# Autodesk Inventor assembly: Ensamble NotAFarmBot2
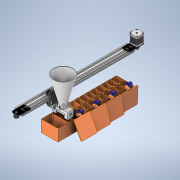
[picture p0: Inventor's stored thumbnail of the model, 180x180]
Saved by Autodesk Inventor 2022 (Build 260153000, 153)
## iProperties
Created: 2020-07-22
Part Number: Ensamble NotAFarmBot2
Document SubType Name: Assembly
Designer: juanp
Mass: 2768.3 g
Surface Area: 9738.48 cm^2
Volume: 1823.12 cm^3
Density: 1.51844 g/cm^3
Author: juanp
## Documents named in this file (24)
- C:\Users\juanp\OneDrive - Universidad de los andes\Uniandes\Robocol\EVA\V0  (Antiguo)\Ensamble NotAFarmBot2.iam
- C:\Users\juanp\OneDrive - Universidad de los andes\Uniandes\Robocol\EVA\V0  (Antiguo)\VSLOT 2040 Extrusion.ipt
- C:\Users\juanp\OneDrive - Universidad de los andes\Uniandes\Robocol\EVA\V0  (Antiguo)\Double Tee Nut.ipt
- C:\Users\juanp\OneDrive - Universidad de los andes\Uniandes\Robocol\EVA\V0  (Antiguo)\GT2_30T_5_6.ipt
- C:\Users\juanp\OneDrive - Universidad de los andes\Uniandes\Robocol\EVA\V0  (Antiguo)\Idler Pulley Plate.ipt
- C:\Users\juanp\OneDrive - Universidad de los andes\Uniandes\Robocol\EVA\V0  (Antiguo)\Motor Mount Plate Nema 17.ipt
- C:\Users\juanp\OneDrive - Universidad de los andes\Uniandes\Robocol\EVA\V0  (Antiguo)\NEMA 17 simple\M1173041- NEMA 17.ipt
- C:\Users\juanp\OneDrive - Universidad de los andes\Uniandes\Robocol\EVA\V0  (Antiguo)\Gantry\Inventor\20mm Gantry Set.iam
- C:\Users\juanp\OneDrive - Universidad de los andes\Uniandes\Robocol\EVA\V0  (Antiguo)\3mm Spacer.ipt
- C:\Users\juanp\OneDrive - Universidad de los andes\Uniandes\Robocol\EVA\V0  (Antiguo)\VSLOT Attachments\M5x25 low profile screw.ipt
- C:\Users\juanp\OneDrive - Universidad de los andes\Uniandes\Robocol\EVA\V0  (Antiguo)\VSLOT Attachments\Ball Bearing 625 2RS 5x16x5.ipt
- C:\Users\juanp\OneDrive - Universidad de los andes\Uniandes\Robocol\EVA\V0  (Antiguo)\VSLOT Attachments\1mm 5mm shim.ipt
- C:\Users\juanp\OneDrive - Universidad de los andes\Uniandes\Robocol\EVA\V0  (Antiguo)\VSLOT Attachments\Nylon Spacer 1_8th.ipt
- C:\Users\juanp\OneDrive - Universidad de los andes\Uniandes\Robocol\EVA\V0  (Antiguo)\VSLOT Attachments\idler pulley.ipt
- C:\Users\juanp\OneDrive - Universidad de los andes\Uniandes\Robocol\EVA\V0  (Antiguo)\Gantry\Inventor\M5 Nylock.ipt
- C:\Users\juanp\OneDrive - Universidad de los andes\Uniandes\Robocol\EVA\V0  (Antiguo)\VSLOT Attachments\M5x8 low profile screw.ipt
- C:\Users\juanp\Documents\Inventor\Content Center Files\R2020\en-US\ANSI B18.3.4M(1)\ANSI B18.3.4M - M3 x 0.5 x 8(2).ipt
- C:\Users\juanp\OneDrive - Universidad de los andes\Uniandes\Robocol\EVA\V0  (Antiguo)\Dispensador V2\Ensamble Dispensador V2.iam
- C:\Users\juanp\OneDrive - Universidad de los andes\Uniandes\Robocol\EVA\V0  (Antiguo)\Gantry\Inventor\M5x35 low profile screw.ipt
- C:\Users\juanp\Documents\Inventor\Content Center Files\R2020\en-US\ANSI B18.3.1M(6)\ANSI B18.3.1M - M2x0.4 x 16(1).ipt
- C:\Users\juanp\Documents\Inventor\Content Center Files\R2020\en-US\ANSI B 18.2.4.1 M(1)\ANSI B 18.2.4.1 M - M2 x 0.4Style 1.ipt
- C:\Users\juanp\OneDrive - Universidad de los andes\Uniandes\Robocol\EVA\V0  (Antiguo)\Tapas.ipt
- C:\Users\juanp\OneDrive - Universidad de los andes\Uniandes\Robocol\EVA\V0  (Antiguo)\SERVO\SG90 - Micro Servo 9g - Tower Pro.iam
- C:\Users\juanp\OneDrive - Universidad de los andes\Uniandes\Robocol\EVA\V0  (Antiguo)\Contenedor3.ipt
## Components (44 placed, 23 different names)
1. VSLOT 2040 Extrusion:1 — Angle:5, Angle:6, Tangent:1, Tangent:2, Mate:85, Mate:86, Mate:87, Mate:88, Angle:16, Mate:98, Mate:99, Angle:18, Mate:100, Mate:101, Angle:23, Angle:24, Flush:3, Mate:180
2. Double Tee Nut:1 — Mate:98, Mate:99, Angle:18, Mate:100, Mate:106
3. Double Tee Nut:2 — Mate:85, Mate:86, Mate:87, Mate:93, Angle:16, Mate:94
4. GT2_30T_5_6:2 — Mate:35, Mate:107
5. Idler Pulley Plate:1 — Mate:88, Mate:89, Mate:90, Mate:91, Mate:92, Mate:95, Mate:96, Mate:97, Angle:17
6. Motor Mount Plate Nema 17:1 — Mate:12, Mate:13, Angle:4, Mate:42, Mate:43, Mate:52, Mate:53, Mate:54, Mate:55, Mate:56, Mate:101, Mate:102, Mate:103, Mate:104, Mate:105
7. M1173041- NEMA 17:1 — Mate:12, Mate:13, Angle:4, Mate:48, Mate:49, Mate:50, Mate:51, Mate:107
8. 20mm Gantry Set:1 [sub-assembly] — Angle:5, Angle:6, Tangent:1, Tangent:2, Mate:56, Mate:121, Mate:124, Mate:126
9. M5x25 low profile screw:1 — Mate:27, Mate:28, Mate:29, Mate:31, Mate:46, Mate:96
10. Ball Bearing 625 2RS 5x16x5:1 — Mate:22, Mate:23, Mate:24, Mate:26, Mate:32
11. Ball Bearing 625 2RS 5x16x5:2 — Mate:21, Mate:25, Mate:28
12. 1mm 5mm shim:1 — Mate:29, Mate:47, Mate:97
13. Nylon Spacer 1_8th:1 — Mate:23, Mate:24, Mate:25
14. idler pulley:1 — Mate:21, Mate:22, Mate:26, Mate:27, Mate:35
15. 3mm Spacer:1 — Mate:31, Mate:32, Mate:95
16. M5x8 low profile screw:1 — Mate:42, Mate:102, Mate:104
17. M5x8 low profile screw:2 — Mate:43, Mate:103, Mate:105, Mate:106
18. M5x8 low profile screw:3 — Mate:90, Mate:92, Mate:94
19. M5x8 low profile screw:4 — Mate:89, Mate:91, Mate:93
20. M5 Nylock:1 — Mate:46, Mate:47, Angle:17
21. Broached Hexagon Socket Button Head Cap Screw - Metric M3 x 0.5 x 8:1 — Mate:50, Mate:54
22. Broached Hexagon Socket Button Head Cap Screw - Metric M3 x 0.5 x 8:2 — Mate:51, Mate:55
23. Broached Hexagon Socket Button Head Cap Screw - Metric M3 x 0.5 x 8:3 — Mate:49, Mate:52
24. Broached Hexagon Socket Button Head Cap Screw - Metric M3 x 0.5 x 8:4 — Mate:48, Mate:53
25. Ensamble Dispensador V2:1 [sub-assembly] — Mate:121, Mate:123, Mate:125, Mate:127, Mate:128, Mate:129, Mate:130, Mate:131, Mate:132, Mate:137, Mate:138, Angle:19, Angle:20, Mate:139, Mate:140, Mate:141, Mate:142, Mate:143, Mate:144, Angle:21, Angle:22, Mate:181
26. M5x35 low profile screw:1 — Mate:125, Mate:126, Mate:128
27. M5x35 low profile screw:2 — Mate:123, Mate:124, Mate:127
28. Forged Socket Head Cap Screw - Metric M2x0.4 x 16:1 — Mate:129, Mate:132, Mate:133
29. Forged Socket Head Cap Screw - Metric M2x0.4 x 16:2 — Mate:130, Mate:131, Mate:134
30. Hex Nut Metric M2 x 0.4:1 — Mate:135, Mate:144, Angle:22
31. Hex Nut Metric M2 x 0.4:2 — Mate:136, Mate:143, Angle:21
32. Hex Nut Metric M2 x 0.4:3 — Mate:134, Mate:138, Angle:19
33. Hex Nut Metric M2 x 0.4:4 — Mate:133, Mate:137, Angle:20
34. Forged Socket Head Cap Screw - Metric M2x0.4 x 16:3 — Mate:135, Mate:140, Mate:142
35. Forged Socket Head Cap Screw - Metric M2x0.4 x 16:4 — Mate:136, Mate:139, Mate:141
36. Tapas:1 — Mate:152, Mate:153, Mate:179, Flush:4
37. Tapas:2 — Mate:160, Mate:161, Mate:177, Mate:179
38. SG90 - Micro Servo 9g - Tower Pro:1 [sub-assembly] — Mate:152, Mate:153, Mate:164, Mate:165
39. SG90 - Micro Servo 9g - Tower Pro:2 [sub-assembly] — Mate:160, Mate:161, Mate:166, Mate:167
40. Contenedor3:1 — Angle:23, Angle:24, Mate:164, Mate:165, Mate:166, Mate:167, Mate:172, Mate:173, Mate:174, Mate:175, Flush:3, Flush:4, Mate:180, Mate:181
41. Tapas:3 — Mate:178
42. SG90 - Micro Servo 9g - Tower Pro:3 [sub-assembly] — Mate:172, Mate:173
43. Tapas:4 — Mate:177, Mate:178
44. SG90 - Micro Servo 9g - Tower Pro:4 [sub-assembly] — Mate:174, Mate:175
## Relationships (110: Mate 94, Angle 12, Tangent 2, Flush 2)
- Mate:12: Motor Mount Plate Nema 17:1 ↔ M1173041- NEMA 17:1
- Mate:13: Motor Mount Plate Nema 17:1 ↔ M1173041- NEMA 17:1
- Angle:4 (0 deg): Motor Mount Plate Nema 17:1 ↔ M1173041- NEMA 17:1
- Angle:5 (0 deg): VSLOT 2040 Extrusion:1 ↔ 20mm Gantry Set:1
- Angle:6 (0 deg): VSLOT 2040 Extrusion:1 ↔ 20mm Gantry Set:1
- Tangent:1: VSLOT 2040 Extrusion:1 ↔ 20mm Gantry Set:1
- Tangent:2: VSLOT 2040 Extrusion:1 ↔ 20mm Gantry Set:1
- Mate:21: Ball Bearing 625 2RS 5x16x5:2 ↔ idler pulley:1
- Mate:22: Ball Bearing 625 2RS 5x16x5:1 ↔ idler pulley:1
- Mate:23: Ball Bearing 625 2RS 5x16x5:1 ↔ Nylon Spacer 1_8th:1
- Mate:24: Ball Bearing 625 2RS 5x16x5:1 ↔ Nylon Spacer 1_8th:1
- Mate:25: Ball Bearing 625 2RS 5x16x5:2 ↔ Nylon Spacer 1_8th:1
- Mate:26: Ball Bearing 625 2RS 5x16x5:1 ↔ idler pulley:1
- Mate:27: M5x25 low profile screw:1 ↔ idler pulley:1
- Mate:28: M5x25 low profile screw:1 ↔ Ball Bearing 625 2RS 5x16x5:2
- Mate:29: M5x25 low profile screw:1 ↔ 1mm 5mm shim:1
- Mate:31: M5x25 low profile screw:1 ↔ 3mm Spacer:1
- Mate:32: Ball Bearing 625 2RS 5x16x5:1 ↔ 3mm Spacer:1
- Mate:35: GT2_30T_5_6:2 ↔ idler pulley:1
- Mate:42: Motor Mount Plate Nema 17:1 ↔ M5x8 low profile screw:1
- Mate:43: Motor Mount Plate Nema 17:1 ↔ M5x8 low profile screw:2
- Mate:46: M5x25 low profile screw:1 ↔ M5 Nylock:1
- Mate:47: 1mm 5mm shim:1 ↔ M5 Nylock:1
- Mate:48: M1173041- NEMA 17:1 ↔ Broached Hexagon Socket Button Head Cap Screw - Metric M3 x 0.5 x 8:4
- Mate:49: M1173041- NEMA 17:1 ↔ Broached Hexagon Socket Button Head Cap Screw - Metric M3 x 0.5 x 8:3
- Mate:50: M1173041- NEMA 17:1 ↔ Broached Hexagon Socket Button Head Cap Screw - Metric M3 x 0.5 x 8:1
- Mate:51: M1173041- NEMA 17:1 ↔ Broached Hexagon Socket Button Head Cap Screw - Metric M3 x 0.5 x 8:2
- Mate:52: Motor Mount Plate Nema 17:1 ↔ Broached Hexagon Socket Button Head Cap Screw - Metric M3 x 0.5 x 8:3
- Mate:53: Motor Mount Plate Nema 17:1 ↔ Broached Hexagon Socket Button Head Cap Screw - Metric M3 x 0.5 x 8:4
- Mate:54: Motor Mount Plate Nema 17:1 ↔ Broached Hexagon Socket Button Head Cap Screw - Metric M3 x 0.5 x 8:1
- Mate:55: Motor Mount Plate Nema 17:1 ↔ Broached Hexagon Socket Button Head Cap Screw - Metric M3 x 0.5 x 8:2
- Mate:56 (358.09 mm): Motor Mount Plate Nema 17:1 ↔ 20mm Gantry Set:1
- Mate:85: VSLOT 2040 Extrusion:1 ↔ Double Tee Nut:2
- Mate:86 (-10 mm): VSLOT 2040 Extrusion:1 ↔ Double Tee Nut:2
- Mate:87: VSLOT 2040 Extrusion:1 ↔ Double Tee Nut:2
- Mate:88: VSLOT 2040 Extrusion:1 ↔ Idler Pulley Plate:1
- Mate:89: Idler Pulley Plate:1 ↔ M5x8 low profile screw:4
- Mate:90: Idler Pulley Plate:1 ↔ M5x8 low profile screw:3
- Mate:91: Idler Pulley Plate:1 ↔ M5x8 low profile screw:4
- Mate:92: Idler Pulley Plate:1 ↔ M5x8 low profile screw:3
- Mate:93: Double Tee Nut:2 ↔ M5x8 low profile screw:4
- Angle:16 (180 deg): VSLOT 2040 Extrusion:1 ↔ Double Tee Nut:2
- Mate:94: Double Tee Nut:2 ↔ M5x8 low profile screw:3
- Mate:95: Idler Pulley Plate:1 ↔ 3mm Spacer:1
- Mate:96: Idler Pulley Plate:1 ↔ M5x25 low profile screw:1
- Mate:97: Idler Pulley Plate:1 ↔ 1mm 5mm shim:1
- Angle:17 (0 deg): Idler Pulley Plate:1 ↔ M5 Nylock:1
- Mate:98: VSLOT 2040 Extrusion:1 ↔ Double Tee Nut:1
- Mate:99: VSLOT 2040 Extrusion:1 ↔ Double Tee Nut:1
- Angle:18 (0 deg): VSLOT 2040 Extrusion:1 ↔ Double Tee Nut:1
- Mate:100 (-10 mm): VSLOT 2040 Extrusion:1 ↔ Double Tee Nut:1
- Mate:101: VSLOT 2040 Extrusion:1 ↔ Motor Mount Plate Nema 17:1
- Mate:102: Motor Mount Plate Nema 17:1 ↔ M5x8 low profile screw:1
- Mate:103: Motor Mount Plate Nema 17:1 ↔ M5x8 low profile screw:2
- Mate:104: Motor Mount Plate Nema 17:1 ↔ M5x8 low profile screw:1
- Mate:105: Motor Mount Plate Nema 17:1 ↔ M5x8 low profile screw:2
- Mate:106: Double Tee Nut:1 ↔ M5x8 low profile screw:2
- Mate:107: GT2_30T_5_6:2 ↔ M1173041- NEMA 17:1
- Mate:121: 20mm Gantry Set:1 ↔ Ensamble Dispensador V2:1
- Mate:123: Ensamble Dispensador V2:1 ↔ M5x35 low profile screw:2
- Mate:124: 20mm Gantry Set:1 ↔ M5x35 low profile screw:2
- Mate:125: Ensamble Dispensador V2:1 ↔ M5x35 low profile screw:1
- Mate:126: 20mm Gantry Set:1 ↔ M5x35 low profile screw:1
- Mate:127: Ensamble Dispensador V2:1 ↔ M5x35 low profile screw:2
- Mate:128: Ensamble Dispensador V2:1 ↔ M5x35 low profile screw:1
- Mate:129: Ensamble Dispensador V2:1 ↔ Forged Socket Head Cap Screw - Metric M2x0.4 x 16:1
- Mate:130: Ensamble Dispensador V2:1 ↔ Forged Socket Head Cap Screw - Metric M2x0.4 x 16:2
- Mate:131: Ensamble Dispensador V2:1 ↔ Forged Socket Head Cap Screw - Metric M2x0.4 x 16:2
- Mate:132: Ensamble Dispensador V2:1 ↔ Forged Socket Head Cap Screw - Metric M2x0.4 x 16:1
- Mate:133: Forged Socket Head Cap Screw - Metric M2x0.4 x 16:1 ↔ Hex Nut Metric M2 x 0.4:4
- Mate:134: Forged Socket Head Cap Screw - Metric M2x0.4 x 16:2 ↔ Hex Nut Metric M2 x 0.4:3
- Mate:135: Hex Nut Metric M2 x 0.4:1 ↔ Forged Socket Head Cap Screw - Metric M2x0.4 x 16:3
- Mate:136: Hex Nut Metric M2 x 0.4:2 ↔ Forged Socket Head Cap Screw - Metric M2x0.4 x 16:4
- Mate:137: Ensamble Dispensador V2:1 ↔ Hex Nut Metric M2 x 0.4:4
- Mate:138: Ensamble Dispensador V2:1 ↔ Hex Nut Metric M2 x 0.4:3
- Angle:19 (0 deg): Ensamble Dispensador V2:1 ↔ Hex Nut Metric M2 x 0.4:3
- Angle:20 (0 deg): Ensamble Dispensador V2:1 ↔ Hex Nut Metric M2 x 0.4:4
- Mate:139: Ensamble Dispensador V2:1 ↔ Forged Socket Head Cap Screw - Metric M2x0.4 x 16:4
- Mate:140: Ensamble Dispensador V2:1 ↔ Forged Socket Head Cap Screw - Metric M2x0.4 x 16:3
- Mate:141: Ensamble Dispensador V2:1 ↔ Forged Socket Head Cap Screw - Metric M2x0.4 x 16:4
- Mate:142: Ensamble Dispensador V2:1 ↔ Forged Socket Head Cap Screw - Metric M2x0.4 x 16:3
- Mate:143: Ensamble Dispensador V2:1 ↔ Hex Nut Metric M2 x 0.4:2
- Mate:144: Ensamble Dispensador V2:1 ↔ Hex Nut Metric M2 x 0.4:1
- Angle:21 (0 deg): Ensamble Dispensador V2:1 ↔ Hex Nut Metric M2 x 0.4:2
- Angle:22 (0 deg): Ensamble Dispensador V2:1 ↔ Hex Nut Metric M2 x 0.4:1
- Mate:152: Tapas:1 ↔ SG90 - Micro Servo 9g - Tower Pro:1
- Mate:153: Tapas:1 ↔ SG90 - Micro Servo 9g - Tower Pro:1
- Mate:160: Tapas:2 ↔ SG90 - Micro Servo 9g - Tower Pro:2
- Mate:161: Tapas:2 ↔ SG90 - Micro Servo 9g - Tower Pro:2
- Angle:23 (0 deg): VSLOT 2040 Extrusion:1 ↔ Contenedor3:1
- Angle:24 (0 deg): VSLOT 2040 Extrusion:1 ↔ Contenedor3:1
- Mate:164: SG90 - Micro Servo 9g - Tower Pro:1 ↔ Contenedor3:1
- Mate:165: SG90 - Micro Servo 9g - Tower Pro:1 ↔ Contenedor3:1
- Mate:166: SG90 - Micro Servo 9g - Tower Pro:2 ↔ Contenedor3:1
- Mate:167: SG90 - Micro Servo 9g - Tower Pro:2 ↔ Contenedor3:1
- [Mate]: Tapas:3 ↔ SG90 - Micro Servo 9g - Tower Pro:3
- [Mate]: Tapas:3 ↔ SG90 - Micro Servo 9g - Tower Pro:3
- [Mate]: Tapas:4 ↔ SG90 - Micro Servo 9g - Tower Pro:4
- [Mate]: Tapas:4 ↔ SG90 - Micro Servo 9g - Tower Pro:4
- Mate:172: Contenedor3:1 ↔ SG90 - Micro Servo 9g - Tower Pro:3
- Mate:173: Contenedor3:1 ↔ SG90 - Micro Servo 9g - Tower Pro:3
- Mate:174: Contenedor3:1 ↔ SG90 - Micro Servo 9g - Tower Pro:4
- Mate:175: Contenedor3:1 ↔ SG90 - Micro Servo 9g - Tower Pro:4
- Mate:177 (1 mm): Tapas:2 ↔ Tapas:4
- Mate:178 (1 mm): Tapas:3 ↔ Tapas:4
- Mate:179 (1 mm): Tapas:1 ↔ Tapas:2
- Flush:3: VSLOT 2040 Extrusion:1 ↔ Contenedor3:1
- Flush:4: Tapas:1 ↔ Contenedor3:1
- Mate:180 (60 mm): VSLOT 2040 Extrusion:1 ↔ Contenedor3:1
- Mate:181: Ensamble Dispensador V2:1 ↔ Contenedor3:1
## Named parameters: d300_d274 = 0 mm, d301_d275 = 0 mm, d302_d274 = 0 mm, d303_d275 = 0 mm
